# Autodesk Inventor assembly: electronica carcasa
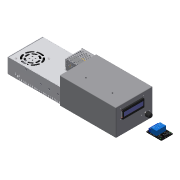
[picture p0: Inventor's stored thumbnail of the model, 180x180]
Saved by Autodesk Inventor 2019 (Build 230136000, 136)
## iProperties
Created: 2019-11-13
Part Number: electronica carcasa
Document SubType Name: Assembly
Designer: Carlos Andres garcia velez
Author: Carlos Andres garcia velez
## Documents named in this file (9)
- C:\Users\user\OneDrive\Carlos_2\02 TRABAJOS\MULTIPLO\Conveyor\ELECTRONICA\electronica carcasa.iam
- C:\Users\user\OneDrive\Carlos_2\02 TRABAJOS\MULTIPLO\Conveyor\ELECTRONICA\LCD.iam
- C:\Users\user\OneDrive\Carlos_2\02 TRABAJOS\MULTIPLO\Conveyor\ELECTRONICA\SMAKN TB6600 STEPPER MOTOR DRIVER.iam
- C:\Users\user\OneDrive\Carlos_2\02 TRABAJOS\MULTIPLO\Conveyor\ELECTRONICA\SCHEDA RELE' 2 CANALI.iam
- C:\Users\user\OneDrive\Carlos_2\02 TRABAJOS\MULTIPLO\Conveyor\ELECTRONICA\Pulse_power_supply_36V_600W.iam
- C:\Users\user\OneDrive\Carlos_2\02 TRABAJOS\MULTIPLO\Conveyor\ELECTRONICA\Power Supply S-60-12 v2.iam
- C:\Users\user\OneDrive\Carlos_2\02 TRABAJOS\MULTIPLO\Conveyor\ELECTRONICA\arduino-nano-shield-cnc-1.snapshot.4 (1)\nano shield.iam
- C:\Users\user\OneDrive\Carlos_2\02 TRABAJOS\MULTIPLO\Conveyor\ELECTRONICA\Rotary Encoder EC11\ROTARY_ENCODER_EC11.iam
- C:\Users\user\OneDrive\Carlos_2\02 TRABAJOS\MULTIPLO\Conveyor\ELECTRONICA\carcasa.ipt
## Components (8 placed, 8 different names)
1. LCD:1 [sub-assembly] — Mate:15, Mate:16, Mate:18
2. SMAKN TB6600 STEPPER MOTOR DRIVER:1 [sub-assembly] — Mate:12, Mate:13, Mate:14
3. SCHEDA RELE' 2 CANALI:1 [sub-assembly]
4. Pulse_power_supply_36V_600W:1 [sub-assembly] — Flush:1, Mate:1, Mate:10, Mate:11, Mate:13
5. Power Supply S-60-12 v2:1 [sub-assembly] — Flush:1, Mate:1, Mate:9
6. nano shield:1 [sub-assembly] — Mate:19, Flush:2, Mate:20
7. ROTARY_ENCODER_EC11:1 [sub-assembly] — Mate:17, Mate:18
8. carcasa:1 — Mate:9, Mate:10, Mate:11, Mate:12, Mate:14, Mate:15, Mate:16, Mate:17, Mate:19, Flush:2, Mate:20
## Relationships (15: Mate 13, Flush 2)
- Flush:1: Pulse_power_supply_36V_600W:1 ↔ Power Supply S-60-12 v2:1
- Mate:1: Pulse_power_supply_36V_600W:1 ↔ Power Supply S-60-12 v2:1
- Mate:9: Power Supply S-60-12 v2:1 ↔ carcasa:1
- Mate:10: Pulse_power_supply_36V_600W:1 ↔ carcasa:1
- Mate:11: Pulse_power_supply_36V_600W:1 ↔ carcasa:1
- Mate:12: SMAKN TB6600 STEPPER MOTOR DRIVER:1 ↔ carcasa:1
- Mate:13 (15 mm): SMAKN TB6600 STEPPER MOTOR DRIVER:1 ↔ Pulse_power_supply_36V_600W:1
- Mate:14 (10 mm): SMAKN TB6600 STEPPER MOTOR DRIVER:1 ↔ carcasa:1
- Mate:15: LCD:1 ↔ carcasa:1
- Mate:16 (5 mm): LCD:1 ↔ carcasa:1
- Mate:17: ROTARY_ENCODER_EC11:1 ↔ carcasa:1
- Mate:18 (5 mm): LCD:1 ↔ ROTARY_ENCODER_EC11:1
- Mate:19 (3 mm): nano shield:1 ↔ carcasa:1
- Flush:2 (8 mm): nano shield:1 ↔ carcasa:1
- Mate:20 (15 mm): nano shield:1 ↔ carcasa:1
